# Autodesk Inventor assembly: FinalRedSail-ver1-1111-2021
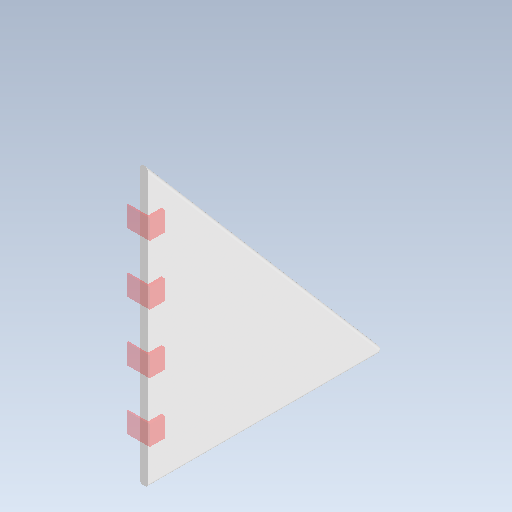
[picture p0: Inventor's stored thumbnail of the model, 512x512]
Saved by Autodesk Inventor 2021 (Build 250183000, 183)
## iProperties
Created: 2021-03-03
Part Number: FinalRedSail-ver1-1111-2021
Document SubType Name: Assembly
Designer: CMurray
Author: CMurray
## Documents named in this file (3)
- F:\PHRC CADD 2021\2021 Game Design Challenge\Sail\Assemblies\FinalRedSail-ver1-1111-2021.iam
- F:\PHRC CADD 2021\2021 Game Design Challenge\Sail\Parts\RedLights-ver-1-1111-2021.ipt
- F:\PHRC CADD 2021\2021 Game Design Challenge\Sail\Parts\RedSail-ver1-1111-2021.ipt
## Components (2 placed, 2 different names)
1. RedLights-ver-1-1111-2021:1 — Mate:1, Flush:2, Mate:2
2. RedSail-ver1-1111-2021:1 — Mate:1, Flush:2, Mate:2
## Relationships (3: Mate 2, Flush 1)
- Mate:1: RedLights-ver-1-1111-2021:1 ↔ RedSail-ver1-1111-2021:1
- Flush:2 (292.1 mm): RedLights-ver-1-1111-2021:1 ↔ RedSail-ver1-1111-2021:1
- Mate:2: RedLights-ver-1-1111-2021:1 ↔ RedSail-ver1-1111-2021:1
